# Autodesk Inventor assembly: Assembly1
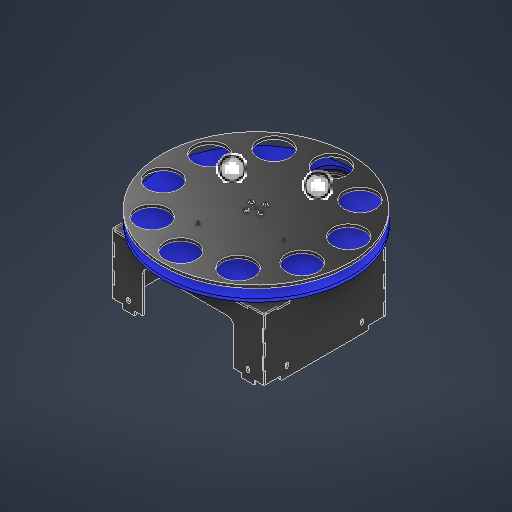
[picture p0: Inventor's stored thumbnail of the model, 512x512]
Saved by Autodesk Inventor 2027.1 (Build 311270010, 270A)
## iProperties
Created: 2026-09-28
Part Number: Assembly1
Document SubType Name: Assembly
Designer: daniel
Author: daniel
## Documents named in this file (17)
- C:\Users\Ahmed\Desktop\Fall 26\Design 1 Repo\MCT333_Design_of_Mechatronics_Systems_1\CAD\FEED and Sorting\Assembly1.iam
- C:\Users\Ahmed\Desktop\Fall 26\Design 1 Repo\MCT333_Design_of_Mechatronics_Systems_1\CAD\FEED and Sorting\Part2.ipt
- C:\Users\Ahmed\Desktop\Fall 26\Design 1 Repo\MCT333_Design_of_Mechatronics_Systems_1\CAD\FEED and Sorting\Part1.ipt
- C:\Users\Ahmed\Desktop\Fall 26\Design 1 Repo\MCT333_Design_of_Mechatronics_Systems_1\CAD\off_the_shelf_components\standard-servo-motor-black-1.snapshot.7\Assem1\Assem1.iam
- C:\Users\Ahmed\Desktop\Fall 26\Design 1 Repo\MCT333_Design_of_Mechatronics_Systems_1\CAD\FEED and Sorting\Part67.ipt
- C:\Users\Ahmed\Desktop\Fall 26\Design 1 Repo\MCT333_Design_of_Mechatronics_Systems_1\CAD\en-US\en-US\GB_T 301-1995(51000)\Rolling bearing 51109 GB_T 301-1995.ipt
- C:\Users\Ahmed\Desktop\Fall 26\Design 1 Repo\MCT333_Design_of_Mechatronics_Systems_1\CAD\FEED and Sorting\Part69.ipt
- C:\Users\Ahmed\Desktop\Fall 26\Design 1 Repo\MCT333_Design_of_Mechatronics_Systems_1\CAD\FEED and Sorting\box\MagazineBox.iam
- C:\Users\Ahmed\Desktop\Fall 26\Design 1 Repo\MCT333_Design_of_Mechatronics_Systems_1\CAD\en-US\en-US\ISO 4032(2)\ISO 4032 - M2.5 - ISO.ipt
- C:\Users\Ahmed\Desktop\Fall 26\Design 1 Repo\MCT333_Design_of_Mechatronics_Systems_1\CAD\fastners\nuts\ANSI B 18.2.4.1 M - M4 x 0.7Style 1.ipt
- C:\Users\Ahmed\Documents\Inventor\Content Center Files\R2027\en-US\ISO 4762(2)\ISO 4762 - M4 x 12ISO.ipt
- C:\Users\SDS Scholar\Documents\Inventor\Content Center Files\R2027\en-US\BS EN ISO 7045 H\EN ISO 7045 - M5 x 20 - 4.8 - H(1).ipt
- C:\Users\Ahmed\Documents\Inventor\Content Center Files\R2027\en-US\ANSI B18.22 M\ANSI B18.22M - 5 N.ipt
- C:\Users\Ahmed\Documents\Inventor\Content Center Files\R2027\en-US\ISO 7045  Z\ISO 7045 - M5 x 20_ - 4.8 - Z - ISO.ipt
- C:\Users\Ahmed\Documents\Inventor\Content Center Files\R2027\en-US\ISO 7045  Z\ISO 7045 - M3 x 20_ - 4.8 - Z - ISO.ipt
- C:\Users\Ahmed\Documents\Inventor\Content Center Files\R2027\en-US\ISO 7045  Z\ISO 7045 - M2.5 x 3_ - 4.8 - Z - ISO.ipt
- C:\Users\Ahmed\Documents\Inventor\Content Center Files\R2027\en-US\ISO 7045  Z\ISO 7045 - M2.5 x 10_ - 4.8 - Z - ISO.ipt
## Components (37 placed, 16 different names)
1. MagazineBox:1 [sub-assembly] — Mate:2, Mate:3, Mate:4, Flush:2, Mate:9, Mate:10, Mate:11, Flush:3, Mate:29, Mate:31
2. Part2:1 — Mate:13, Mate:14, Mate:15, Mate:16, Insert:9, Insert:10, Insert:11, Insert:12, Mate:33, Mate:34, Mate:35, Mate:36, Mate:37, Mate:38, Mate:39, Mate:40, Mate:49, Insert:13, Insert:14, Insert:15, Insert:16, Insert:17, Insert:18, Insert:19, Insert:20, Insert:21, Insert:22
3. Part1:1 — Mate:2, Mate:3, Mate:5, Mate:6, Mate:7, Mate:8, Mate:12
4. Assem1:1 [sub-assembly] — Mate:9, Mate:10, Mate:11, Mate:30, Mate:41, Mate:43, Mate:47, Mate:49
5. Part67:1 — Mate:4, Flush:2, Mate:5, Flush:3
6. Rolling bearing GB/T 301-1995 Type 51000 51109:1 — Mate:12, Tangent:1, Tangent:2, Flush:4
7. Part69:1 — Tangent:2, Flush:4, Mate:13, Mate:14, Mate:15, Mate:16
8. Part69:2 — Mate:6, Mate:7, Mate:8, Tangent:1
9. ISO 4032 M2.5:1 — Insert:9
10. ISO 4032 M2.5:2 — Insert:10
11. ISO 4032 M2.5:3 — Insert:11
12. ISO 4032 M2.5:4 — Insert:12
13. BS EN ISO 7045 H - Metric M5 x 20 - 4.8 - H:1 — Mate:34, Mate:38
14. BS EN ISO 7045 H - Metric M5 x 20 - 4.8 - H:2 — Mate:33, Mate:37, Mate:48
15. BS EN ISO 7045 H - Metric M5 x 20 - 4.8 - H:3 — Mate:35, Mate:40, Mate:44
16. BS EN ISO 7045 H - Metric M5 x 20 - 4.8 - H:4 — Mate:36, Mate:39, Mate:42
17. Plain Washer (Metric) 5 N:1 — Mate:47, Mate:48
18. Plain Washer (Metric) 5 N:2 — Mate:43, Mate:44
19. Plain Washer (Metric) 5 N:4 — Mate:41, Mate:42
20. ISO 7045 Z M5 x 20 - 4.8 - Z:3 — Insert:13
21. ISO 7045 Z M5 x 20 - 4.8 - Z:4 — Insert:14
22. ISO 7045 Z M5 x 20 - 4.8 - Z:1 — Insert:15
23. ISO 7045 Z M5 x 20 - 4.8 - Z:2 — Insert:16
24. ISO 7045 Z M3 x 20 - 4.8 - Z:1 — Insert:17
25. ISO 7045 Z M2.5 x 10 - 4.8 - Z:1 — Insert:18
26. ISO 7045 Z M2.5 x 3 - 4.8 - Z:2 — Insert:19
27. ISO 7045 Z M2.5 x 10 - 4.8 - Z:2 — Insert:20
28. ISO 7045 Z M2.5 x 10 - 4.8 - Z:4 — Insert:21
29. ISO 7045 Z M2.5 x 10 - 4.8 - Z:3 — Insert:22
30. ISO 4762 M4 x 12:1 — Mate:29, Mate:30, Mate:32
31. Hex Nut Metric M4 x 0.7:1 — Mate:31, Mate:32
32. ISO 4762 M4 x 12:2
33. Hex Nut Metric M4 x 0.7:2
34. ISO 4762 M4 x 12:3
35. Hex Nut Metric M4 x 0.7:3
36. ISO 4762 M4 x 12:4
37. Hex Nut Metric M4 x 0.7:4
## Component patterns: (4 elements, first: ISO 4762 M4 x 12:1 + Hex Nut Metric M4 x 0.7:1)
## Relationships (53: Mate 34, Insert 14, Flush 3, Tangent 2)
- Mate:2: MagazineBox:1 ↔ Part1:1
- Mate:3: MagazineBox:1 ↔ Part1:1
- Mate:4: MagazineBox:1 ↔ Part67:1
- Flush:2: MagazineBox:1 ↔ Part67:1
- Mate:5: Part1:1 ↔ Part67:1
- Mate:6: Part1:1 ↔ Part69:2
- Mate:7: Part1:1 ↔ Part69:2
- Mate:8: Part1:1 ↔ Part69:2
- Mate:9: MagazineBox:1 ↔ Assem1:1
- Mate:10: MagazineBox:1 ↔ Assem1:1
- Mate:11: MagazineBox:1 ↔ Assem1:1
- Mate:12: Part1:1 ↔ Rolling bearing GB/T 301-1995 Type 51000 51109:1
- Tangent:1: Rolling bearing GB/T 301-1995 Type 51000 51109:1 ↔ Part69:2
- Tangent:2: Rolling bearing GB/T 301-1995 Type 51000 51109:1 ↔ Part69:1
- Flush:3: MagazineBox:1 ↔ Part67:1
- Flush:4: Rolling bearing GB/T 301-1995 Type 51000 51109:1 ↔ Part69:1
- Mate:13: Part2:1 ↔ Part69:1
- Mate:14: Part2:1 ↔ Part69:1
- Mate:15: Part2:1 ↔ Part69:1
- Mate:16: Part2:1 ↔ Part69:1
- Insert:9: Part2:1 ↔ ISO 4032 M2.5:1
- Insert:10: Part2:1 ↔ ISO 4032 M2.5:2
- Insert:11: Part2:1 ↔ ISO 4032 M2.5:3
- Insert:12: Part2:1 ↔ ISO 4032 M2.5:4
- Mate:29: MagazineBox:1 ↔ ISO 4762 M4 x 12:1
- Mate:30: Assem1:1 ↔ ISO 4762 M4 x 12:1
- Mate:31: MagazineBox:1 ↔ Hex Nut Metric M4 x 0.7:1
- Mate:32: ISO 4762 M4 x 12:1 ↔ Hex Nut Metric M4 x 0.7:1
- Mate:33: Part2:1 ↔ BS EN ISO 7045 H - Metric M5 x 20 - 4.8 - H:2
- Mate:34: Part2:1 ↔ BS EN ISO 7045 H - Metric M5 x 20 - 4.8 - H:1
- Mate:35: Part2:1 ↔ BS EN ISO 7045 H - Metric M5 x 20 - 4.8 - H:3
- Mate:36: Part2:1 ↔ BS EN ISO 7045 H - Metric M5 x 20 - 4.8 - H:4
- Mate:37: Part2:1 ↔ BS EN ISO 7045 H - Metric M5 x 20 - 4.8 - H:2
- Mate:38: Part2:1 ↔ BS EN ISO 7045 H - Metric M5 x 20 - 4.8 - H:1
- Mate:39: Part2:1 ↔ BS EN ISO 7045 H - Metric M5 x 20 - 4.8 - H:4
- Mate:40: Part2:1 ↔ BS EN ISO 7045 H - Metric M5 x 20 - 4.8 - H:3
- Mate:41: Assem1:1 ↔ Plain Washer (Metric) 5 N:4
- Mate:42: BS EN ISO 7045 H - Metric M5 x 20 - 4.8 - H:4 ↔ Plain Washer (Metric) 5 N:4
- Mate:43: Assem1:1 ↔ Plain Washer (Metric) 5 N:2
- Mate:44: BS EN ISO 7045 H - Metric M5 x 20 - 4.8 - H:3 ↔ Plain Washer (Metric) 5 N:2
- Mate:47: Assem1:1 ↔ Plain Washer (Metric) 5 N:1
- Mate:48: BS EN ISO 7045 H - Metric M5 x 20 - 4.8 - H:2 ↔ Plain Washer (Metric) 5 N:1
- Mate:49: Part2:1 ↔ Assem1:1
- Insert:13: Part2:1 ↔ ISO 7045 Z M5 x 20 - 4.8 - Z:3
- Insert:14: Part2:1 ↔ ISO 7045 Z M5 x 20 - 4.8 - Z:4
- Insert:15: Part2:1 ↔ ISO 7045 Z M5 x 20 - 4.8 - Z:1
- Insert:16: Part2:1 ↔ ISO 7045 Z M5 x 20 - 4.8 - Z:2
- Insert:17: Part2:1 ↔ ISO 7045 Z M3 x 20 - 4.8 - Z:1
- Insert:18: Part2:1 ↔ ISO 7045 Z M2.5 x 10 - 4.8 - Z:1
- Insert:19: Part2:1 ↔ ISO 7045 Z M2.5 x 3 - 4.8 - Z:2
- Insert:20: Part2:1 ↔ ISO 7045 Z M2.5 x 10 - 4.8 - Z:2
- Insert:21: Part2:1 ↔ ISO 7045 Z M2.5 x 10 - 4.8 - Z:4
- Insert:22: Part2:1 ↔ ISO 7045 Z M2.5 x 10 - 4.8 - Z:3
